# Autodesk Inventor assembly: RODA MONTADA
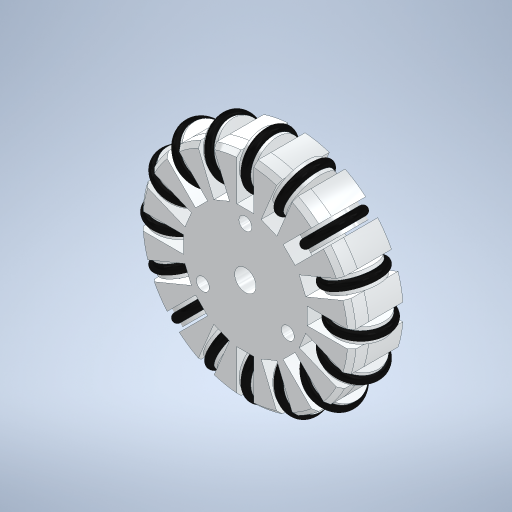
[picture p0: Inventor's stored thumbnail of the model, 512x512]
Saved by Autodesk Inventor 2023 (Build 270158000, 158)
## iProperties
Created: 2009-10-15
Part Number: RODA MONTADA
Document SubType Name: Assembly
Designer: leonardo.saglio
Sending System: SolidWorks 2016
Last Author: Ocelus
Last Saved: 2017-07-17
Author: leonardo.saglio
## Documents named in this file (5)
- C:\Users\hiago.sodre\Downloads\Model_2XL430-W250-T\Roda nova\RODA MONTADA.iam
- C:\Users\hiago.sodre\Downloads\Model_2XL430-W250-T\Roda nova\roda1.ipt
- C:\Users\hiago.sodre\Downloads\Model_2XL430-W250-T\Roda nova\RODA 2 MODIFICADA.ipt
- C:\Users\hiago.sodre\Downloads\Model_2XL430-W250-T\Roda nova\rollers.ipt
- C:\Users\hiago.sodre\Downloads\Model_2XL430-W250-T\Roda nova\orings.ipt
## Components (4 placed, 4 different names)
1. roda1:1 — De rotación:1
2. RODA 2 MODIFICADA:1 — De rotación:1, Rígido:2
3. rollers:1 — Rígido:1, Rígido:2
4. orings:1 — Rígido:1
## Relationships (3: WeldJoint 2, RevoluteJoint 1)
- De rotación:1 [RevoluteJoint]: roda1:1 ↔ RODA 2 MODIFICADA:1
- Rígido:1 [WeldJoint]: rollers:1 ↔ orings:1
- Rígido:2 [WeldJoint]: RODA 2 MODIFICADA:1 ↔ rollers:1
